# Autodesk Inventor assembly: 部件1
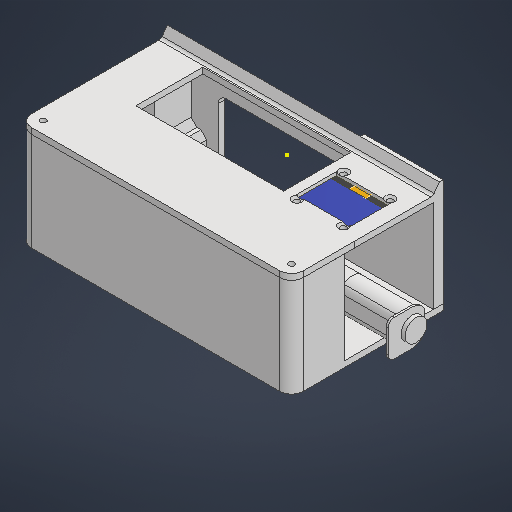
[picture p0: Inventor's stored thumbnail of the model, 512x512]
Saved by Autodesk Inventor 2025 (Build 290162000, 162)
## iProperties
Created: 2025-11-30
Part Number: 部件1
Document SubType Name: Assembly
Designer: XH
Author: XH
## Documents named in this file (13)
- C:\1A_Engineering_files\braille-printer-v2\部件1.iam
- C:\1A_Engineering_files\braille-printer-v2\便签.ipt
- C:\1A_Engineering_files\braille-printer-v2\主体.ipt
- C:\1A_Engineering_files\braille-printer-v2\针头主体.iam
- C:\1A_Engineering_files\braille-printer-v2\钢轴.ipt
- C:\1A_Engineering_files\braille-printer-v2\Y轴杠轴.ipt
- C:\1A_Engineering_files\braille-printer-v2\xy转接连杆.ipt
- C:\1A_Engineering_files\braille-printer-v2\阻挡X轴.ipt
- C:\1A_Engineering_files\braille-printer-v2\大外壳.ipt
- C:\1A_Engineering_files\braille-printer-v2\电机.ipt
- C:\1A_Engineering_files\braille-printer-v2\后盖电路.ipt
- C:\1A_Engineering_files\braille-printer-v2\前舵机位置控制.ipt
- C:\1A_Engineering_files\braille-printer-v2\Weewooday I2C OLED 0.96'' 128x64.iam
## Components (13 placed, 12 different names)
1. 便签:1 — 配合:1, 配合:2
2. 主体:1 — 配合:1, 配合:2, 表面齐平:7, 配合:12, 配合:19, 表面齐平:10, 表面齐平:11, 配合:23, 配合:26, 表面齐平:12, 表面齐平:13, 配合:27, 配合:28, 配合:29
3. 针头主体:1 [sub-assembly] — 配合:4, 配合:5
4. 钢轴:1 — 表面齐平:3, 配合:4, 配合:6, 配合:10
5. 钢轴:2 — 表面齐平:3, 配合:5, 配合:7, 表面齐平:8, 配合:11
6. Y轴杠轴:2 — 配合:9, 配合:12
7. xy转接连杆:1 — 配合:6, 配合:7, 表面齐平:7, 配合:9, 配合:22
8. 阻挡X轴:1 — 表面齐平:8, 配合:10, 配合:11
9. 大外壳:1 — 配合:19, 表面齐平:10, 表面齐平:11, 配合:25
10. 电机:1 — 配合:22, 配合:23
11. 后盖电路:1 — 配合:25
12. 前舵机位置控制:1 — 配合:26, 表面齐平:12, 表面齐平:13
13. Weewooday I2C OLED 0.96'' 128x64:1 [sub-assembly] — 配合:27, 配合:28, 配合:29
## Relationships (25: Mate 18, Flush 7)
- 配合:1 [Mate]: 便签:1 ↔ 主体:1
- 配合:2 [Mate]: 便签:1 ↔ 主体:1
- 表面齐平:3 [Flush]: 钢轴:1 ↔ 钢轴:2
- 配合:4 [Mate]: 针头主体:1 ↔ 钢轴:1
- 配合:5 [Mate]: 针头主体:1 ↔ 钢轴:2
- 配合:6 [Mate]: 钢轴:1 ↔ xy转接连杆:1
- 配合:7 [Mate]: 钢轴:2 ↔ xy转接连杆:1
- 表面齐平:7 [Flush]: 主体:1 ↔ xy转接连杆:1
- 配合:9 [Mate]: Y轴杠轴:2 ↔ xy转接连杆:1
- 表面齐平:8 [Flush]: 钢轴:2 ↔ 阻挡X轴:1
- 配合:10 [Mate]: 钢轴:1 ↔ 阻挡X轴:1
- 配合:11 [Mate]: 钢轴:2 ↔ 阻挡X轴:1
- 配合:12 [Mate]: 主体:1 ↔ Y轴杠轴:2
- 配合:19 [Mate]: 主体:1 ↔ 大外壳:1
- 表面齐平:10 [Flush]: 主体:1 ↔ 大外壳:1
- 表面齐平:11 [Flush]: 主体:1 ↔ 大外壳:1
- 配合:22 [Mate]: xy转接连杆:1 ↔ 电机:1
- 配合:23 [Mate]: 主体:1 ↔ 电机:1
- 配合:25 [Mate]: 大外壳:1 ↔ 后盖电路:1
- 配合:26 [Mate]: 主体:1 ↔ 前舵机位置控制:1
- 表面齐平:12 [Flush]: 主体:1 ↔ 前舵机位置控制:1
- 表面齐平:13 [Flush]: 主体:1 ↔ 前舵机位置控制:1
- 配合:27 [Mate]: 主体:1 ↔ Weewooday I2C OLED 0.96'' 128x64:1
- 配合:28 [Mate]: 主体:1 ↔ Weewooday I2C OLED 0.96'' 128x64:1
- 配合:29 [Mate]: 主体:1 ↔ Weewooday I2C OLED 0.96'' 128x64:1
